# Autodesk Inventor assembly: RobotFab Frame 3
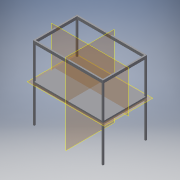
[picture p0: Inventor's stored thumbnail of the model, 180x180]
Saved by Autodesk Inventor 2019 (Build 230136000, 136)
## iProperties
Created: 2021-05-09
Part Number: RobotFab Frame 3
Document SubType Name: Assembly
Designer: Eric
Author: Eric
## Documents named in this file (10)
- C:\Users\Eric\Documents\! - Uni\Year 4\MENG-Robot-Fab-Project\Models\For_Optimiser\RobotFab Frame 3.iam
- C:\Users\Eric\Documents\! - Uni\Year 4\MENG-Robot-Fab-Project\Models\For_Optimiser\RobotFabFrame_1.ipt
- C:\Users\Eric\Documents\! - Uni\Year 4\MENG-Robot-Fab-Project\Models\For_Optimiser\RobotFabFrame_2.ipt
- C:\Users\Eric\Documents\! - Uni\Year 4\MENG-Robot-Fab-Project\Models\For_Optimiser\RobotFabFrame_3.ipt
- C:\Users\Eric\Documents\! - Uni\Year 4\MENG-Robot-Fab-Project\Models\For_Optimiser\RobotFabFrame_4.ipt
- C:\Users\Eric\Documents\! - Uni\Year 4\MENG-Robot-Fab-Project\Models\For_Optimiser\RobotFabFrame_5.ipt
- C:\Users\Eric\Documents\! - Uni\Year 4\MENG-Robot-Fab-Project\Models\For_Optimiser\RobotFabFrame_6.ipt
- C:\Users\Eric\Documents\! - Uni\Year 4\MENG-Robot-Fab-Project\Models\For_Optimiser\RobotFabFrame_7.ipt
- C:\Users\Eric\Documents\! - Uni\Year 4\MENG-Robot-Fab-Project\Models\For_Optimiser\RobotFabFrame_8.ipt
- C:\Users\Eric\Documents\! - Uni\Year 4\MENG-Robot-Fab-Project\Models\For_Optimiser\RobotFabFrame_9.ipt
## Components (9 placed, 9 different names)
1. RobotFabFrame_1:1 — Symmetry:1
2. RobotFabFrame_2:1 — Symmetry:2
3. RobotFabFrame_3:1 — Symmetry:3
4. RobotFabFrame_4:1 — Symmetry:2
5. RobotFabFrame_5:1 — Symmetry:3
6. RobotFabFrame_6:1
7. RobotFabFrame_7:1
8. RobotFabFrame_8:1
9. RobotFabFrame_9:1 — Symmetry:1
## Relationships (3: Symmetry 3)
- Symmetry:1: RobotFabFrame_1:1 ↔ RobotFabFrame_9:1
- Symmetry:2: RobotFabFrame_2:1 ↔ RobotFabFrame_4:1
- Symmetry:3: RobotFabFrame_3:1 ↔ RobotFabFrame_5:1
